# Autodesk Inventor assembly: assembly edited 2
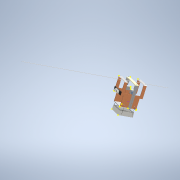
[picture p0: Inventor's stored thumbnail of the model, 180x180]
Saved by Autodesk Inventor 2021.3 (Build 253353010, 353A)
## iProperties
Created: 2021-07-07
Part Number: assembly edited 2
Document SubType Name: Assembly
Designer: VK
Author: VK
## Documents named in this file (15)
- D:\C CYCLE\Autodesk Inventor\Exploration\assembly edited 2.iam
- D:\C CYCLE\Autodesk Inventor\Exploration\part1 edited.ipt
- D:\C CYCLE\Autodesk Inventor\Exploration\motor(1 shaft).ipt
- D:\C CYCLE\Autodesk Inventor\Exploration\Part6.ipt
- D:\C CYCLE\Autodesk Inventor\Exploration\part3.ipt
- D:\C CYCLE\Autodesk Inventor\Exploration\Part2.ipt
- D:\C CYCLE\Autodesk Inventor\Exploration\part 2 upper part.ipt
- D:\C CYCLE\Autodesk Inventor\Exploration\bottom part.ipt
- D:\C CYCLE\Autodesk Inventor\Exploration\container 1.ipt
- D:\C CYCLE\Autodesk Inventor\Exploration\ir sensor stand.ipt
- D:\C CYCLE\Autodesk Inventor\Exploration\ir sensor.ipt
- D:\C CYCLE\Autodesk Inventor\Exploration\screw.ipt
- D:\C CYCLE\Autodesk Inventor\Exploration\bulb edited.ipt
- D:\C CYCLE\Autodesk Inventor\Exploration\battery.ipt
- D:\C CYCLE\Autodesk Inventor\Exploration\square rope.ipt
## Components (24 placed, 14 different names)
1. part1 edited:1 — Mate:1, Flush:1, Flush:2, Mate:2, Flush:3, Flush:4, Mate:4, Flush:7, Flush:8, Mate:18, Flush:16, Mate:20, Flush:18, Flush:19, Mate:28, Tangent:1
2. motor(1 shaft):1 — Mate:1, Flush:1, Flush:2, Rotational:2
3. part1 edited:2 — Mate:3, Flush:5, Flush:6, Mate:5, Flush:9, Flush:10, Mate:16, Mate:17, Mate:19, Flush:15, Flush:17, Mate:21, Mate:25, Mate:26, Mate:30
4. Part6:1 — Mate:2, Flush:3, Flush:4, Mate:3, Flush:5, Flush:6
5. Part6:2 — Mate:4, Flush:7, Flush:8, Slider:1, Rotation:1
6. motor(1 shaft):2 — Mate:5, Flush:9, Flush:10, Mate:37, Mate:38
7. bottom part:1 — Mate:16, Mate:17, Mate:18, Mate:19, Flush:15, Flush:16, Flush:17, Mate:27, Flush:21, Mate:29
8. container 1:1
9. ir sensor stand:1 — Mate:20, Mate:21, Flush:18, Flush:19, Mate:22, Flush:20, Mate:23, Mate:24
10. ir sensor:1 — Mate:22, Flush:20, Mate:31, Mate:32
11. screw:1 — Mate:23
12. screw:2 — Mate:24
13. bulb edited:1 — Mate:25
14. bulb edited:2 — Mate:26
15. battery:1 — Mate:29, Mate:30
16. battery:2 — Mate:27, Mate:28, Flush:21
17. screw:3 — Mate:31
18. screw:4 — Mate:32
19. part3:3 — Rotational:2, Mate:35, Mate:36
20. Part2:1 — Mate:35, Mate:36, Tangent:1, Mate:42, Flush:22, Flush:23
21. part3:4 — Mate:37, Mate:38
22. part 2 upper part:1 — Mate:42, Flush:22, Flush:23, Mate:43, Flush:24, Flush:25
23. Part2:2 — Mate:43, Flush:24, Flush:25
24. square rope:1 — Slider:1, Rotation:1
## Relationships (53: Mate 28, Flush 21, RevoluteJoint 1, Tangent 1, TranslationJoint 1, RelateRotation 1)
- Mate:1: part1 edited:1 ↔ motor(1 shaft):1
- Flush:1: part1 edited:1 ↔ motor(1 shaft):1
- Flush:2: part1 edited:1 ↔ motor(1 shaft):1
- Mate:2: part1 edited:1 ↔ Part6:1
- Flush:3: part1 edited:1 ↔ Part6:1
- Flush:4: part1 edited:1 ↔ Part6:1
- Mate:3: part1 edited:2 ↔ Part6:1
- Flush:5: part1 edited:2 ↔ Part6:1
- Flush:6: part1 edited:2 ↔ Part6:1
- Mate:4: part1 edited:1 ↔ Part6:2
- Flush:7: part1 edited:1 ↔ Part6:2
- Flush:8: part1 edited:1 ↔ Part6:2
- Mate:5: part1 edited:2 ↔ motor(1 shaft):2
- Flush:9: part1 edited:2 ↔ motor(1 shaft):2
- Flush:10: part1 edited:2 ↔ motor(1 shaft):2
- Mate:16: part1 edited:2 ↔ bottom part:1
- Mate:17: part1 edited:2 ↔ bottom part:1
- Mate:18: part1 edited:1 ↔ bottom part:1
- Mate:19: part1 edited:2 ↔ bottom part:1
- Flush:15: part1 edited:2 ↔ bottom part:1
- Flush:16: part1 edited:1 ↔ bottom part:1
- Flush:17: part1 edited:2 ↔ bottom part:1
- Mate:20: part1 edited:1 ↔ ir sensor stand:1
- Mate:21: part1 edited:2 ↔ ir sensor stand:1
- Flush:18: part1 edited:1 ↔ ir sensor stand:1
- Flush:19: part1 edited:1 ↔ ir sensor stand:1
- Mate:22: ir sensor stand:1 ↔ ir sensor:1
- Flush:20: ir sensor stand:1 ↔ ir sensor:1
- Mate:23: ir sensor stand:1 ↔ screw:1
- Mate:24: ir sensor stand:1 ↔ screw:2
- Mate:25: part1 edited:2 ↔ bulb edited:1
- Mate:26: part1 edited:2 ↔ bulb edited:2
- Mate:27: bottom part:1 ↔ battery:2
- Mate:28: part1 edited:1 ↔ battery:2
- Flush:21: bottom part:1 ↔ battery:2
- Mate:29: bottom part:1 ↔ battery:1
- Mate:30: part1 edited:2 ↔ battery:1
- Mate:31: ir sensor:1 ↔ screw:3
- Mate:32: ir sensor:1 ↔ screw:4
- Rotational:2 [RevoluteJoint] (-10 mm): motor(1 shaft):1 ↔ part3:3
- Mate:35: part3:3 ↔ Part2:1
- Mate:36: part3:3 ↔ Part2:1
- Tangent:1: part1 edited:1 ↔ Part2:1
- Mate:37: motor(1 shaft):2 ↔ part3:4
- Mate:38: motor(1 shaft):2 ↔ part3:4
- Mate:42: Part2:1 ↔ part 2 upper part:1
- Flush:22: Part2:1 ↔ part 2 upper part:1
- Flush:23: Part2:1 ↔ part 2 upper part:1
- Mate:43: part 2 upper part:1 ↔ Part2:2
- Flush:24: part 2 upper part:1 ↔ Part2:2
- Flush:25: part 2 upper part:1 ↔ Part2:2
- Slider:1 [TranslationJoint]: Part6:2 ↔ square rope:1
- Rotation:1 [RelateRotation] (1 ul): Part6:2 ↔ square rope:1
